# Autodesk Inventor assembly: config - motherboard - single processor
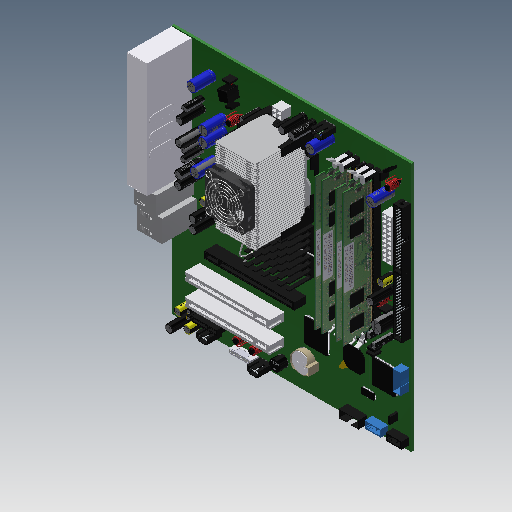
[picture p0: Inventor's stored thumbnail of the model, 512x512]
Saved by Autodesk Inventor 2020 (Build 240152000, 152)
## iProperties
Created: 2005-12-05
Part Number: config - motherboard - single processor
Document SubType Name: Assembly
Designer: Simon.Ng@autodesk.com
Stock Number: NA
Description: Control Board
Mass: 476.849 g
Surface Area: 5141.45 cm^2
Volume: 476.849 cm^3
Density: 1 g/cm^3
Company: Autodesk Asia Pte. Ltd.
Title: In House Assembly
Author: Simon.Ng@autodesk.com
Revision Number: A
## Documents named in this file (36)
- C:\Users\hallc\Desktop\Process Equipment\Workspace\Supplier Content\Electrical Design\Motherboard\Motherboard.iam
- C:\Users\hallc\Desktop\Process Equipment\Workspace\Supplier Content\Electrical Design\Motherboard\J9B1 Connector.ipt
- C:\Users\hallc\Desktop\Process Equipment\Workspace\Supplier Content\Electrical Design\Motherboard\J9C2 Connector.ipt
- C:\Users\hallc\Desktop\Process Equipment\Workspace\Supplier Content\Electrical Design\Motherboard\PCIE Connector.ipt
- C:\Users\hallc\Desktop\Process Equipment\Workspace\Supplier Content\Electrical Design\Motherboard\C9G5 connector.ipt
- C:\Users\hallc\Desktop\Process Equipment\Workspace\Supplier Content\Electrical Design\Motherboard\J9H2 Connector.ipt
- C:\Users\hallc\Desktop\Process Equipment\Workspace\Supplier Content\Electrical Design\Motherboard\PCI Slot.ipt
- C:\Users\hallc\Desktop\Process Equipment\Workspace\Supplier Content\Electrical Design\Motherboard\AGP slot.ipt
- C:\Users\hallc\Desktop\Process Equipment\Workspace\Supplier Content\Electrical Design\Motherboard\DDR Connector.ipt
- C:\Users\hallc\Desktop\Process Equipment\Workspace\Supplier Content\Electrical Design\Motherboard\RJ45 Module.ipt
- C:\Users\hallc\Desktop\Process Equipment\Workspace\Supplier Content\Electrical Design\Motherboard\USB Module.ipt
- C:\Users\hallc\Desktop\Process Equipment\Workspace\Supplier Content\Electrical Design\Motherboard\IO Interface Module.ipt
- C:\Users\hallc\Desktop\Process Equipment\Workspace\Supplier Content\Electrical Design\Motherboard\Capacitor 1000 UF.ipt
- C:\Users\hallc\Desktop\Process Equipment\Workspace\Supplier Content\Electrical Design\Motherboard\Capacitor 560 UF.ipt
- C:\Users\hallc\Desktop\Process Equipment\Workspace\Supplier Content\Electrical Design\Motherboard\Capacitor 1200 UF.ipt
- C:\Users\hallc\Desktop\Process Equipment\Workspace\Supplier Content\Electrical Design\Motherboard\Capacitor 640 UF.ipt
- C:\Users\hallc\Desktop\Process Equipment\Workspace\Supplier Content\Electrical Design\Motherboard\Capacitor 3000 UF.ipt
- C:\Users\hallc\Desktop\Process Equipment\Workspace\Supplier Content\Electrical Design\Motherboard\Choke.ipt
- C:\Users\hallc\Desktop\Process Equipment\Workspace\Supplier Content\Electrical Design\Motherboard\Battery.ipt
- C:\Users\hallc\Desktop\Process Equipment\Workspace\Supplier Content\Electrical Design\Motherboard\Bezel.ipt
- C:\Users\hallc\Desktop\Process Equipment\Workspace\Supplier Content\Electrical Design\Motherboard\Chip 15 x15.ipt
- C:\Users\hallc\Desktop\Process Equipment\Workspace\Supplier Content\Electrical Design\Motherboard\Capacitor 3500 UF.ipt
- C:\Users\hallc\Desktop\Process Equipment\Workspace\Supplier Content\Electrical Design\Motherboard\Chip block.ipt
- C:\Users\hallc\Desktop\Process Equipment\Workspace\Supplier Content\Electrical Design\Motherboard\Chip stand.ipt
- C:\Users\hallc\Desktop\Process Equipment\Workspace\Supplier Content\Electrical Design\Motherboard\Chip 13 x 6.ipt
- C:\Users\hallc\Desktop\Process Equipment\Workspace\Supplier Content\Electrical Design\Motherboard\Chip 22 x 11.ipt
- C:\Users\hallc\Desktop\Process Equipment\Workspace\Supplier Content\Electrical Design\Motherboard\Chip 24 x 23.ipt
- C:\Users\hallc\Desktop\Process Equipment\Workspace\Supplier Content\Electrical Design\Motherboard\RAM - DDR.ipt
- C:\Users\hallc\Desktop\Process Equipment\Workspace\Supplier Content\Electrical Design\Motherboard\Motherboard Heat Sink.ipt
- C:\Users\hallc\Desktop\Process Equipment\Workspace\Supplier Content\Electrical Design\Motherboard\IDE Male Connector.ipt
- C:\Users\hallc\Desktop\Process Equipment\Workspace\Supplier Content\Electrical Design\Motherboard\Processor Heat Sink Mounting.ipt
- C:\Users\hallc\Desktop\Process Equipment\Workspace\Supplier Content\Electrical Design\Motherboard\Processor Heat Sink.ipt
- C:\Users\hallc\Desktop\Process Equipment\Workspace\Supplier Content\Electrical Design\Motherboard\Processor Fan\Cooling Fan, 40mm x 40mm x 10 mm, 12VDC.iam
- C:\Users\hallc\Desktop\Process Equipment\Workspace\Supplier Content\Electrical Design\Motherboard\Power Supply Header 2.ipt
- C:\Users\hallc\Desktop\Process Equipment\Workspace\Supplier Content\Electrical Design\Motherboard\Power Supply Header 1.ipt
- C:\Users\hallc\Desktop\Process Equipment\Workspace\Supplier Content\Electrical Design\Motherboard\Motherboard PCB (Tyler).ipt
## Components (111 placed, 35 different names)
1. PCI Slot:3
2. Motherboard PCB (Tyler):1 — Mate:84, Mate:85, Mate:86, Mate:87, Mate:88, Mate:89
3. J9B1 Connector:1
4. J9B1 Connector:2
5. J9C2 Connector:1
6. PCIE Connector:1
7. C9G5 connector:1
8. J9H2 Connector:1
9. J9H2 Connector:2
10. C9G5 connector:2
11. IDE Male Connector:1
12. IDE Male Connector:2
13. Power Supply Header 1:1 — Mate:84, Mate:85, Mate:86
14. J9B1 Connector:3
15. AGP slot:1
16. Processor Heat Sink Mounting:1
17. Processor Heat Sink:1 — Mate:83, Flush:18, Flush:19
18. RJ45 Module:1
19. USB Module:1
20. IO Interface Module:1
21. Capacitor 560 UF:1
22. Capacitor 1200 UF:1
23. Capacitor 560 UF:2
24. Capacitor 640 UF:1
25. Capacitor 640 UF:2
26. Capacitor 1000 UF:2
27. Capacitor 3000 UF:1
28. Capacitor 1200 UF:2
29. Capacitor 560 UF:8
30. Capacitor 560 UF:9
31. Capacitor 560 UF:10
32. Capacitor 560 UF:11
33. Capacitor 560 UF:12
34. Capacitor 3000 UF:2
35. Capacitor 3000 UF:3
36. Capacitor 3000 UF:4
37. Capacitor 3000 UF:5
38. Capacitor 560 UF:13
39. Capacitor 560 UF:14
40. Capacitor 1200 UF:3
41. Capacitor 1200 UF:4
42. Capacitor 1200 UF:5
43. Capacitor 640 UF:8
44. Capacitor 640 UF:9
45. Capacitor 640 UF:10
46. Capacitor 640 UF:11
47. Capacitor 640 UF:12
48. Capacitor 640 UF:13
49. Capacitor 3000 UF:6
50. Capacitor 560 UF:16
51. Capacitor 1200 UF:6
52. Capacitor 1200 UF:7
53. Capacitor 1200 UF:8
54. Capacitor 3000 UF:7
55. Choke:1
56. Choke:2
57. Choke:3
58. Battery:1
59. Bezel:1
60. Chip 15 x15:1
61. Capacitor 3500 UF:1
62. Capacitor 1000 UF:5
63. Capacitor 1000 UF:6
64. Capacitor 1200 UF:9
65. Capacitor 1200 UF:11
66. Capacitor 1200 UF:10
67. Capacitor 1200 UF:12
68. Capacitor 1000 UF:7
69. Capacitor 1000 UF:8
70. Capacitor 1000 UF:9
71. Chip block:1
72. Chip block:2
73. Chip block:3
74. Chip stand:1 — Flush:13
75. Chip stand:2 — Flush:9, Flush:10
76. Chip stand:3 — Flush:8, Flush:9
77. Chip stand:4 — Flush:7, Flush:8
78. Chip stand:5 — Flush:11, Flush:12, Flush:13
79. Chip stand:6 — Flush:16, Flush:17
80. Chip stand:7 — Flush:12
81. Chip stand:8 — Flush:6, Flush:7, Flush:10, Flush:11
82. Chip stand:9 — Flush:5, Flush:6
83. Chip stand:10 — Flush:5, Flush:17
84. Chip stand:11 — Flush:15, Flush:16
85. Chip stand:12 — Flush:14
86. Chip stand:13 — Flush:14, Flush:15
87. Chip 13 x 6:1
88. Chip 13 x 6:2
89. Chip 13 x 6:3
90. Chip 22 x 11:1
91. Chip 22 x 11:3
92. Chip 24 x 23:1
93. Chip 24 x 23:2
94. Choke:4
95. Choke:5
96. Choke:6
97. Choke:7
98. Capacitor 560 UF:17
99. Motherboard Heat Sink:1
100. Cooling Fan, 40mm x 40mm x 10 mm, 12VDC:1 [sub-assembly] — Mate:83, Flush:18, Flush:19
101. Power Supply Header 2:1 — Mate:87, Mate:88, Mate:89
102. PCI Slot:1
103. PCI Slot:2
104. DDR Connector:1 — Mate:80, Mate:81, Mate:82
105. DDR Connector:2
106. DDR Connector:3
107. DDR Connector:4
108. RAM - DDR:1 — Mate:80, Mate:81, Mate:82
109. RAM - DDR:2
110. RAM - DDR:3
111. RAM - DDR:4
## Component patterns: (2 elements, first: PCI Slot:1), (5 elements, first: DDR Connector:1), (5 elements, first: RAM - DDR:1)
## Relationships (25: Flush 15, Mate 10)
- Flush:5: Chip stand:9 ↔ Chip stand:10
- Flush:6: Chip stand:8 ↔ Chip stand:9
- Flush:7: Chip stand:4 ↔ Chip stand:8
- Flush:8: Chip stand:3 ↔ Chip stand:4
- Flush:9: Chip stand:2 ↔ Chip stand:3
- Flush:10: Chip stand:2 ↔ Chip stand:8
- Flush:11: Chip stand:5 ↔ Chip stand:8
- Flush:12: Chip stand:5 ↔ Chip stand:7
- Flush:13: Chip stand:1 ↔ Chip stand:5
- Flush:14: Chip stand:12 ↔ Chip stand:13
- Flush:15: Chip stand:11 ↔ Chip stand:13
- Flush:16: Chip stand:6 ↔ Chip stand:11
- Flush:17: Chip stand:6 ↔ Chip stand:10
- Mate:80: DDR Connector:1 ↔ RAM - DDR:1
- Mate:81 (2.5 mm): DDR Connector:1 ↔ RAM - DDR:1
- Mate:82 (0.5 mm): DDR Connector:1 ↔ RAM - DDR:1
- Mate:83: Processor Heat Sink:1 ↔ Cooling Fan, 40mm x 40mm x 10 mm, 12VDC:1
- Flush:18 (17.25 mm): Processor Heat Sink:1 ↔ Cooling Fan, 40mm x 40mm x 10 mm, 12VDC:1
- Flush:19: Processor Heat Sink:1 ↔ Cooling Fan, 40mm x 40mm x 10 mm, 12VDC:1
- Mate:84: Motherboard PCB (Tyler):1 ↔ Power Supply Header 1:1
- Mate:85: Motherboard PCB (Tyler):1 ↔ Power Supply Header 1:1
- Mate:86: Motherboard PCB (Tyler):1 ↔ Power Supply Header 1:1
- Mate:87: Motherboard PCB (Tyler):1 ↔ Power Supply Header 2:1
- Mate:88: Motherboard PCB (Tyler):1 ↔ Power Supply Header 2:1
- Mate:89: Motherboard PCB (Tyler):1 ↔ Power Supply Header 2:1
